# Autodesk Inventor assembly: SUBWashThrustArm
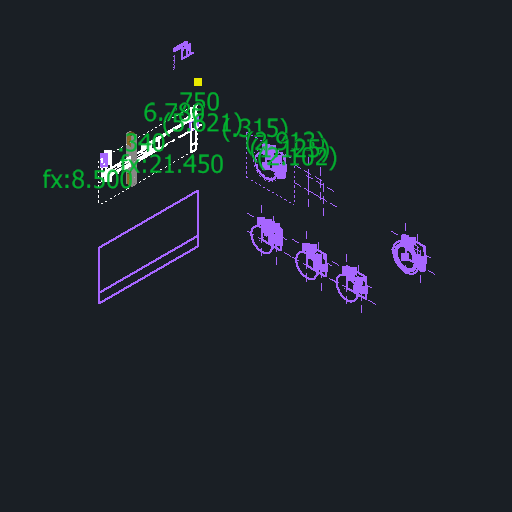
[picture p0: Inventor's stored thumbnail of the model, 512x512]
Saved by Autodesk Inventor 2024 (Build 280153000, 153)
## iProperties
Created: 2025-02-08
Part Number: SUBWashThrustArm
Document SubType Name: Assembly
Designer: Tommy Rohmann
Author: Tommy Rohmann
## Documents named in this file (4)
- C:\Users\Tommy Rohmann\OneDrive\Projects\Microgravity-Press-Washing-Machine\System Design and Documentation\Inventor Design Project\SUBWashThrustArm.iam
- C:\Users\Tommy Rohmann\OneDrive\Projects\Microgravity-Press-Washing-Machine\System Design and Documentation\Inventor Design Project\LAYOUT.ipt
- C:\Users\Tommy Rohmann\OneDrive\Projects\Microgravity-Press-Washing-Machine\System Design and Documentation\Inventor Design Project\ACMEThrustNut.ipt
- C:\Users\Tommy Rohmann\OneDrive\Projects\Microgravity-Press-Washing-Machine\System Design and Documentation\Inventor Design Project\ThrustArmWash.ipt
## Components (7 placed, 3 different names)
1. LAYOUT:1
2. ACMEThrustNut:1 — Mate:1, Flush:1, Flush:2, Flush:3, Flush:4, Mate:8
3. ThrustArmWash:1 — Mate:1, Mate:2, Mate:3, Mate:4, Flush:1, Flush:2, Flush:5, Flush:6
4. ThrustArmWash:2 — Mate:2, Mate:3, Mate:4
5. ThrustArmWash:3
6. ThrustArmWash:4 — Flush:3, Flush:4, Mate:8, Mate:9
7. ACMEThrustNut:2 — Flush:5, Mate:9, Flush:6
## Relationships (17: Mate 9, Flush 6, Composite 2)
- [Composite]: LAYOUT:1 ↔ ACMEThrustNut:1
- [Composite]: LAYOUT:1 ↔ ThrustArmWash:1
- Mate:1: ACMEThrustNut:1 ↔ ThrustArmWash:1
- Mate:2: ThrustArmWash:1 ↔ ThrustArmWash:2
- Mate:3: ThrustArmWash:1 ↔ ThrustArmWash:2
- Mate:4: ThrustArmWash:1 ↔ ThrustArmWash:2
- Flush:1: ACMEThrustNut:1 ↔ ThrustArmWash:1
- Flush:2: ACMEThrustNut:1 ↔ ThrustArmWash:1
- [Mate]: ThrustArmWash:3 ↔ ThrustArmWash:4
- [Mate]: ThrustArmWash:3 ↔ ThrustArmWash:4
- [Mate]: ThrustArmWash:3 ↔ ThrustArmWash:4
- Flush:3: ACMEThrustNut:1 ↔ ThrustArmWash:4
- Flush:4: ACMEThrustNut:1 ↔ ThrustArmWash:4
- Mate:8: ACMEThrustNut:1 ↔ ThrustArmWash:4
- Flush:5: ThrustArmWash:1 ↔ ACMEThrustNut:2
- Mate:9: ThrustArmWash:4 ↔ ACMEThrustNut:2
- Flush:6: ThrustArmWash:1 ↔ ACMEThrustNut:2
## Named parameters: d14_d9 = 0 mm, d15_d10 = 0 mm, d16_d11 = 0 mm
